# Autodesk Inventor assembly: A2017_T2_13
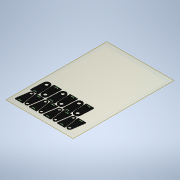
[picture p0: Inventor's stored thumbnail of the model, 180x180]
Saved by Autodesk Inventor 2020 (Build 240168000, 168)
## iProperties
Created: 2021-08-27
Part Number: A2017_T2_13
Document SubType Name: Assembly
Designer: Masato
Author: Masato
## Documents named in this file (4)
- D:\GitHub\inventor\SUSTAINA-OP\Cam\A2017_T2_13.iam
- D:\GitHub\inventor\SUSTAINA-OP\Cam\DisposableBoard.ipt
- D:\GitHub\inventor\SUSTAINA-OP\LowerBody\Foot\Foot_front_frame.ipt
- D:\GitHub\inventor\SUSTAINA-OP\LowerBody\Foot\Foot_back_frame.ipt
## Components (15 placed, 3 different names)
1. DisposableBoard:1 — メイト:2, メイト:1, フラッシュ:1, フラッシュ:2, メイト:4, メイト:5, メイト:6, メイト:7, 正接:1, メイト:9, メイト:10, メイト:13
2. Foot_front_frame:2 — メイト:7, メイト:8, 正接:1, 正接:3
3. Foot_front_frame:1 — メイト:4, メイト:5, メイト:6, メイト:8, 正接:2
4. Foot_front_frame:3
5. Foot_front_frame:4
6. Foot_front_frame:5
7. Foot_front_frame:6
8. Foot_front_frame:7
9. Foot_front_frame:8
10. Foot_back_frame:1 — メイト:10, メイト:14, 正接:3
11. Foot_back_frame:2 — メイト:9, 正接:2, メイト:13, メイト:14
12. Foot_back_frame:3
13. Foot_back_frame:4
14. Foot_back_frame:5
15. Foot_back_frame:6
## Component patterns: (4 elements, first: Foot_front_frame:2 + Foot_front_frame:1), (3 elements, first: Foot_back_frame:1 + Foot_back_frame:2)
## Relationships (16: Mate 11, Tangent 3, Flush 2)
- メイト:2 [Mate]: DisposableBoard:1
- メイト:1 [Mate]: DisposableBoard:1
- フラッシュ:1 [Flush]: DisposableBoard:1
- フラッシュ:2 [Flush]: DisposableBoard:1
- メイト:4 [Mate]: DisposableBoard:1 ↔ Foot_front_frame:1
- メイト:5 [Mate] (2 mm): DisposableBoard:1 ↔ Foot_front_frame:1
- メイト:6 [Mate] (2 mm): DisposableBoard:1 ↔ Foot_front_frame:1
- メイト:7 [Mate]: DisposableBoard:1 ↔ Foot_front_frame:2
- メイト:8 [Mate] (2.5 mm): Foot_front_frame:2 ↔ Foot_front_frame:1
- 正接:1 [Tangent] (2 mm): DisposableBoard:1 ↔ Foot_front_frame:2
- メイト:9 [Mate]: DisposableBoard:1 ↔ Foot_back_frame:2
- メイト:10 [Mate]: DisposableBoard:1 ↔ Foot_back_frame:1
- 正接:2 [Tangent] (2.5 mm): Foot_front_frame:1 ↔ Foot_back_frame:2
- メイト:13 [Mate] (2 mm): DisposableBoard:1 ↔ Foot_back_frame:2
- メイト:14 [Mate] (2.5 mm): Foot_back_frame:1 ↔ Foot_back_frame:2
- 正接:3 [Tangent] (2.5 mm): Foot_front_frame:2 ↔ Foot_back_frame:1
